# Autodesk Inventor assembly: PCB
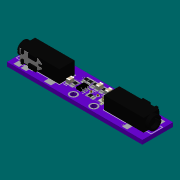
[picture p0: Inventor's stored thumbnail of the model, 180x180]
Saved by Autodesk Inventor 2016 (Build 200138000, 138)
## iProperties
Created: 2015-08-25
Part Number: PCB
Document SubType Name: Assembly
Designer: Cosmic
Author: Cosmic
## Documents named in this file (8)
- C:\Users\Sawaiz\Documents\3d\inventor\mppcSensorInterface\sensorV3.iam
- C:\Users\Sawaiz\Documents\3d\inventor\mppcSensorInterface\electronics\SJ-4351X-SMT.ipt
- C:\Users\Sawaiz\Documents\3d\inventor\mppcSensorInterface\electronics\128-0711-201.ipt
- C:\Users\Sawaiz\Documents\3d\inventor\mppcSensorInterface\electronics\MPPC.ipt
- C:\Users\Sawaiz\Documents\3d\inventor\mppcSensorInterface\electronics\0805.ipt
- C:\Users\Sawaiz\Documents\3d\inventor\mppcSensorInterface\electronics\0805 Capacitor.ipt
- C:\Users\Sawaiz\Documents\3d\inventor\mppcSensorInterface\electronics\SOT23_5.ipt
- C:\Users\Sawaiz\Documents\3d\inventor\mppcSensorInterface\pcbV3.ipt
## Components (16 placed, 7 different names)
1. pcbV3:1 — Mate:1, Mate:2, Mate:3, Mate:4, Mate:5, Mate:6, Mate:7, Mate:8, Mate:9, Angle:9, Angle:10
2. SJ-4351X-SMT:1 — Flush:1, Mate:9, Angle:9
3. SJ-4351X-SMT:2 — Flush:1, Mate:7, Mate:8, Angle:10
4. 128-0711-201:1 — Mate:5
5. MPPC:1 — Mate:1, Mate:2, Mate:3
6. 0805:1 — Flush:7, Mate:6
7. 0805:3 — Flush:4, Flush:5, Flush:7, Flush:8
8. 0805:5 — Flush:5, Flush:6, Flush:8, Flush:9
9. 0805:6 — Flush:2, Flush:3, Flush:9, Flush:10
10. 0805:7 — Flush:6, Flush:10
11. 0805:8 — Flush:2, Flush:13, Flush:14
12. 0805:9 — Flush:3, Flush:4
13. 0805 Capacitor:1 — Flush:11, Flush:12, Angle:7, Angle:8
14. 0805 Capacitor:2 — Flush:11, Angle:7, Flush:13, Mate:4
15. 0805 Capacitor:3 — Flush:12, Angle:8
16. SOT23_5:1 — Flush:14
## Relationships (27: Flush 14, Mate 9, Angle 4)
- Flush:1: SJ-4351X-SMT:1 ↔ SJ-4351X-SMT:2
- Flush:2: 0805:6 ↔ 0805:8
- Flush:3: 0805:6 ↔ 0805:9
- Flush:4: 0805:3 ↔ 0805:9
- Flush:5: 0805:3 ↔ 0805:5
- Flush:6: 0805:5 ↔ 0805:7
- Flush:7: 0805:1 ↔ 0805:3
- Flush:8: 0805:3 ↔ 0805:5
- Flush:9: 0805:5 ↔ 0805:6
- Flush:10: 0805:6 ↔ 0805:7
- Flush:11: 0805 Capacitor:1 ↔ 0805 Capacitor:2
- Flush:12: 0805 Capacitor:1 ↔ 0805 Capacitor:3
- Angle:7 (0 deg): 0805 Capacitor:1 ↔ 0805 Capacitor:2
- Angle:8 (0 deg): 0805 Capacitor:1 ↔ 0805 Capacitor:3
- Mate:1: pcbV3:1 ↔ MPPC:1
- Mate:2: pcbV3:1 ↔ MPPC:1
- Mate:3: pcbV3:1 ↔ MPPC:1
- Flush:13: 0805:8 ↔ 0805 Capacitor:2
- Flush:14: 0805:8 ↔ SOT23_5:1
- Mate:4: pcbV3:1 ↔ 0805 Capacitor:2
- Mate:5: pcbV3:1 ↔ 128-0711-201:1
- Mate:6: pcbV3:1 ↔ 0805:1
- Mate:7: pcbV3:1 ↔ SJ-4351X-SMT:2
- Mate:8: pcbV3:1 ↔ SJ-4351X-SMT:2
- Mate:9: pcbV3:1 ↔ SJ-4351X-SMT:1
- Angle:9 (0 deg): pcbV3:1 ↔ SJ-4351X-SMT:1
- Angle:10 (0 deg): pcbV3:1 ↔ SJ-4351X-SMT:2
